# Autodesk Inventor assembly: Assembly2
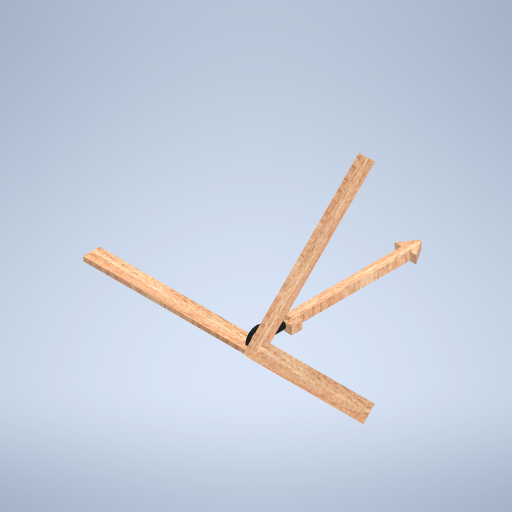
[picture p0: Inventor's stored thumbnail of the model, 512x512]
Saved by Autodesk Inventor 2023 (Build 270158000, 158)
## iProperties
Created: 2023-11-27
Part Number: Assembly2
Document SubType Name: Assembly
Designer: Mustapha
Author: Mustapha
## Documents named in this file (6)
- D:\EDU\Senior 2\Robotics\Activity\SideProject\Assembly2.iam
- D:\EDU\Senior 2\Robotics\Activity\SideProject\Zaxix.ipt
- D:\EDU\Senior 2\Robotics\Activity\SideProject\OriginNutipt.ipt
- D:\EDU\Senior 2\Robotics\Activity\SideProject\Vector.ipt
- D:\EDU\Senior 2\Robotics\Activity\SideProject\Yaxix.ipt
- D:\EDU\Senior 2\Robotics\Activity\SideProject\Xaxix .ipt
## Components (5 placed, 5 different names)
1. Zaxix:1 — Mate:3, Mate:4, Flush:2
2. OriginNutipt:1 — Flush:2, Mate:5, Mate:6, Mate:7
3. Vector:1 — Mate:6, Mate:7
4. Yaxix:1 — Mate:1, Mate:2, Flush:1, Mate:5
5. Xaxix :2 — Mate:1, Mate:2, Mate:3, Flush:1, Mate:4
## Relationships (9: Mate 7, Flush 2)
- Mate:1: Yaxix:1 ↔ Xaxix :2
- Mate:2: Yaxix:1 ↔ Xaxix :2
- Mate:3: Zaxix:1 ↔ Xaxix :2
- Flush:1: Yaxix:1 ↔ Xaxix :2
- Mate:4: Zaxix:1 ↔ Xaxix :2
- Flush:2 (30 mm): Zaxix:1 ↔ OriginNutipt:1
- Mate:5 (5 mm): OriginNutipt:1 ↔ Yaxix:1
- Mate:6: OriginNutipt:1 ↔ Vector:1
- Mate:7 (-12 mm): OriginNutipt:1 ↔ Vector:1
